# Autodesk Inventor assembly: Weapon Assembly
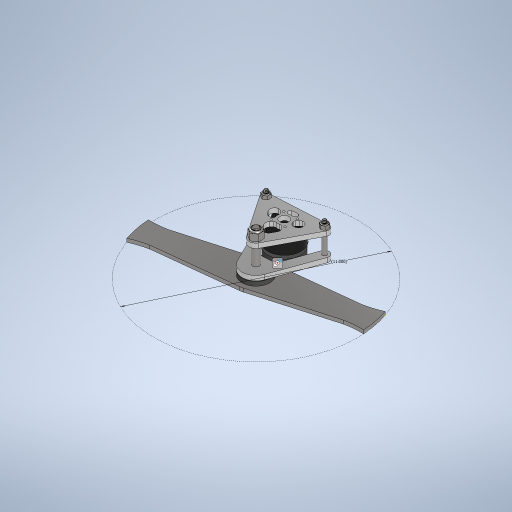
[picture p0: Inventor's stored thumbnail of the model, 512x512]
Saved by Autodesk Inventor 2023.1 (Build 271208000, 208)
## iProperties
Created: 2022-05-21
Part Number: Weapon Assembly
Document SubType Name: Assembly
Designer: Nathan Cai
Mass: 726.994 g
Surface Area: 717.319 cm^2
Volume: 134.119 cm^3
Density: 5.42049 g/cm^3
Author: Nathan Cai
## Documents named in this file (9)
- E:\Documents\Inventor\0.3rd Lawette - V3.4\Horizontal Weapon Assembly (Type U)\Weapon Assembly (Horizontal U).iam
- E:\Documents\Inventor\0.3rd Lawette - V3.4\Horizontal Weapon Assembly (Type U)\Weapon (Weapon-Side Pulley).iam
- E:\Documents\Inventor\0.3rd Lawette - V3.4\Horizontal Weapon Assembly (Type U)\90807A139_Same-Size Thread Alloy Steel Shoulder Screw.ipt
- E:\Documents\Inventor\0.3rd Lawette - V3.4\Horizontal Weapon Assembly (Type U)\90630A121_High-Strength Steel Nylon-Insert Locknut.ipt
- E:\Documents\Inventor\0.3rd Lawette - V3.4\Horizontal Weapon Assembly (Type U)\Weapon (Motor-Side Pulley).iam
- E:\Documents\Inventor\0.3rd Lawette - V3.4\Horizontal Weapon Assembly (Type U)\Frame (Clear Side).ipt
- E:\Documents\Inventor\0.3rd Lawette - V3.4\Horizontal Weapon Assembly (Type U)\Frame (Motor Side).ipt
- E:\Documents\Inventor\0.3rd Lawette - V3.4\Horizontal Weapon Assembly (Type U)\90969A180_Ultra-Low-Profile Shoulder Screw.ipt
- E:\Documents\Inventor\0.3rd Lawette - V3.4\Horizontal Weapon Assembly (Type U)\91831A011_18-8 Stainless Steel Nylon-Insert Locknut.ipt
## Components (10 placed, 8 different names)
1. Weapon (Weapon-Side Pulley):1 [sub-assembly] — Mate:174, Mate:191
2. 90807A139_Same-Size Thread Alloy Steel Shoulder Screw:1 — Mate:1, Mate:2, Mate:9, Mate:174
3. 90630A121_High-Strength Steel Nylon-Insert Locknut:1 — Mate:1, Mate:2, Mate:173
4. Frame (Motor Side):1 — Symmetry:1, Mate:173, Mate:177, Mate:183, Mate:184, Mate:187, Mate:188, Mate:189, Mate:190
5. Frame (Clear Side):1 — Mate:9, Symmetry:1, Mate:176, Mate:178, Mate:179, Mate:180, Mate:187, Mate:191
6. Weapon (Motor-Side Pulley):1 [sub-assembly] — Mate:188, Mate:189, Mate:190
7. 90969A180_Ultra-Low-Profile Shoulder Screw:1 — Mate:176, Mate:177, Mate:178, Mate:181
8. 90969A180_Ultra-Low-Profile Shoulder Screw:2 — Mate:179, Mate:180, Mate:182
9. 91831A011_18-8 Stainless Steel Nylon-Insert Locknut:1 — Mate:182, Mate:184
10. 91831A011_18-8 Stainless Steel Nylon-Insert Locknut:2 — Mate:181, Mate:183
## Relationships (22: Mate 21, Symmetry 1)
- Mate:1: 90807A139_Same-Size Thread Alloy Steel Shoulder Screw:1 ↔ 90630A121_High-Strength Steel Nylon-Insert Locknut:1
- Mate:2 (50.8 mm): 90807A139_Same-Size Thread Alloy Steel Shoulder Screw:1 ↔ 90630A121_High-Strength Steel Nylon-Insert Locknut:1
- [Mate]: 90807A139_Same-Size Thread Alloy Steel Shoulder Screw:1 ↔ Frame (Motor Side):1
- Mate:9: 90807A139_Same-Size Thread Alloy Steel Shoulder Screw:1 ↔ Frame (Clear Side):1
- [Mate]: Frame (Motor Side):1 ↔ Frame (Clear Side):1
- Symmetry:1: Frame (Motor Side):1 ↔ Frame (Clear Side):1
- Mate:173: 90630A121_High-Strength Steel Nylon-Insert Locknut:1 ↔ Frame (Motor Side):1
- Mate:174: Weapon (Weapon-Side Pulley):1 ↔ 90807A139_Same-Size Thread Alloy Steel Shoulder Screw:1
- Mate:176: Frame (Clear Side):1 ↔ 90969A180_Ultra-Low-Profile Shoulder Screw:1
- Mate:177: Frame (Motor Side):1 ↔ 90969A180_Ultra-Low-Profile Shoulder Screw:1
- Mate:178: Frame (Clear Side):1 ↔ 90969A180_Ultra-Low-Profile Shoulder Screw:1
- Mate:179: Frame (Clear Side):1 ↔ 90969A180_Ultra-Low-Profile Shoulder Screw:2
- Mate:180: Frame (Clear Side):1 ↔ 90969A180_Ultra-Low-Profile Shoulder Screw:2
- Mate:181: 90969A180_Ultra-Low-Profile Shoulder Screw:1 ↔ 91831A011_18-8 Stainless Steel Nylon-Insert Locknut:2
- Mate:182: 90969A180_Ultra-Low-Profile Shoulder Screw:2 ↔ 91831A011_18-8 Stainless Steel Nylon-Insert Locknut:1
- Mate:183: Frame (Motor Side):1 ↔ 91831A011_18-8 Stainless Steel Nylon-Insert Locknut:2
- Mate:184: Frame (Motor Side):1 ↔ 91831A011_18-8 Stainless Steel Nylon-Insert Locknut:1
- Mate:187 (25.4 mm): Frame (Motor Side):1 ↔ Frame (Clear Side):1
- Mate:188: Frame (Motor Side):1 ↔ Weapon (Motor-Side Pulley):1
- Mate:189: Frame (Motor Side):1 ↔ Weapon (Motor-Side Pulley):1
- Mate:190: Frame (Motor Side):1 ↔ Weapon (Motor-Side Pulley):1
- Mate:191: Weapon (Weapon-Side Pulley):1 ↔ Frame (Clear Side):1
